# Autodesk Inventor assembly: 40mm Gantry Set universal
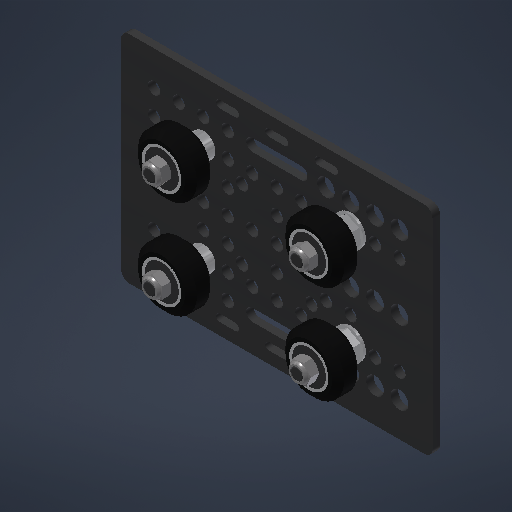
[picture p0: Inventor's stored thumbnail of the model, 512x512]
Saved by Autodesk Inventor 2027.1 (Build 311270010, 270A)
## iProperties
Created: 2016-04-11
Part Number: 40mm Gantry Set universal
Document SubType Name: Assembly
Designer: Ben
Author: Ben
## Documents named in this file (6)
- E:\Apps\AutodeskInventor\University\MCT333_Design1\OnTheShelf\VSoltGantrySetAllSizes\Inventor\40mm Gantry Set universal.iam
- E:\Apps\AutodeskInventor\University\MCT333_Design1\OnTheShelf\VSoltGantrySetAllSizes\Inventor\80mm gantry plate.ipt
- E:\Apps\AutodeskInventor\University\MCT333_Design1\OnTheShelf\VSoltGantrySetAllSizes\Inventor\V-Wheel Solid Wheel.iam
- E:\Apps\AutodeskInventor\University\MCT333_Design1\OnTheShelf\VSoltGantrySetAllSizes\Inventor\V-Wheel Solid Wheel - spacer.iam
- E:\Apps\AutodeskInventor\University\MCT333_Design1\OnTheShelf\VSoltGantrySetAllSizes\Inventor\M5x25 low profile screw.ipt
- E:\Apps\AutodeskInventor\University\MCT333_Design1\OnTheShelf\VSoltGantrySetAllSizes\Inventor\M5 Nylock.ipt
## Components (13 placed, 5 different names)
1. 80mm gantry plate:1 — Mate:3, Mate:4, Mate:5, Mate:6, Mate:7, Mate:8, Mate:9, Mate:10, Mate:13, Mate:14, Mate:15, Mate:16, Flush:1, Flush:2, Flush:3, Flush:4, Flush:5
2. V-Wheel Solid Wheel:1 [sub-assembly] — Mate:5, Mate:8, Mate:11, Mate:23
3. V-Wheel Solid Wheel:2 [sub-assembly] — Mate:6, Mate:7, Mate:12, Mate:24
4. V-Wheel Solid Wheel - spacer:1 [sub-assembly] — Mate:2, Mate:3, Mate:21
5. V-Wheel Solid Wheel - spacer:2 [sub-assembly] — Mate:1, Mate:4, Mate:22
6. M5x25 low profile screw:1 — Mate:10, Mate:16, Mate:20, Mate:2
7. M5x25 low profile screw:2 — Mate:9, Mate:15, Mate:19, Mate:1
8. M5x25 low profile screw:3 — Mate:11, Mate:14, Mate:18
9. M5x25 low profile screw:4 — Mate:12, Mate:13, Mate:17
10. M5 Nylock:1 — Mate:20, Mate:21
11. M5 Nylock:2 — Mate:19, Mate:22
12. M5 Nylock:3 — Mate:18, Mate:23
13. M5 Nylock:4 — Mate:17, Mate:24
## Relationships (30: Mate 24, Flush 6)
- Mate:1: V-Wheel Solid Wheel - spacer:2 ↔ M5x25 low profile screw:2
- Mate:2: V-Wheel Solid Wheel - spacer:1 ↔ M5x25 low profile screw:1
- Mate:3: 80mm gantry plate:1 ↔ V-Wheel Solid Wheel - spacer:1
- Mate:4: 80mm gantry plate:1 ↔ V-Wheel Solid Wheel - spacer:2
- Mate:5: 80mm gantry plate:1 ↔ V-Wheel Solid Wheel:1
- Mate:6: 80mm gantry plate:1 ↔ V-Wheel Solid Wheel:2
- Mate:7: 80mm gantry plate:1 ↔ V-Wheel Solid Wheel:2
- Mate:8: 80mm gantry plate:1 ↔ V-Wheel Solid Wheel:1
- Mate:9: 80mm gantry plate:1 ↔ M5x25 low profile screw:2
- Mate:10: 80mm gantry plate:1 ↔ M5x25 low profile screw:1
- Mate:11: V-Wheel Solid Wheel:1 ↔ M5x25 low profile screw:3
- Mate:12: V-Wheel Solid Wheel:2 ↔ M5x25 low profile screw:4
- Mate:13: 80mm gantry plate:1 ↔ M5x25 low profile screw:4
- Mate:14: 80mm gantry plate:1 ↔ M5x25 low profile screw:3
- Mate:15: 80mm gantry plate:1 ↔ M5x25 low profile screw:2
- Mate:16: 80mm gantry plate:1 ↔ M5x25 low profile screw:1
- Mate:17: M5x25 low profile screw:4 ↔ M5 Nylock:4
- Mate:18: M5x25 low profile screw:3 ↔ M5 Nylock:3
- Mate:19: M5x25 low profile screw:2 ↔ M5 Nylock:2
- Mate:20: M5x25 low profile screw:1 ↔ M5 Nylock:1
- Mate:21: V-Wheel Solid Wheel - spacer:1 ↔ M5 Nylock:1
- Mate:22: V-Wheel Solid Wheel - spacer:2 ↔ M5 Nylock:2
- Mate:23: V-Wheel Solid Wheel:1 ↔ M5 Nylock:3
- Mate:24: V-Wheel Solid Wheel:2 ↔ M5 Nylock:4
- Flush:1 (11.885 mm): 80mm gantry plate:1
- Flush:2: 80mm gantry plate:1
- Flush:3: 80mm gantry plate:1
- Flush:4: 80mm gantry plate:1
- Flush:5: 80mm gantry plate:1
- Flush:6
